# Autodesk Inventor assembly: Inner_Components
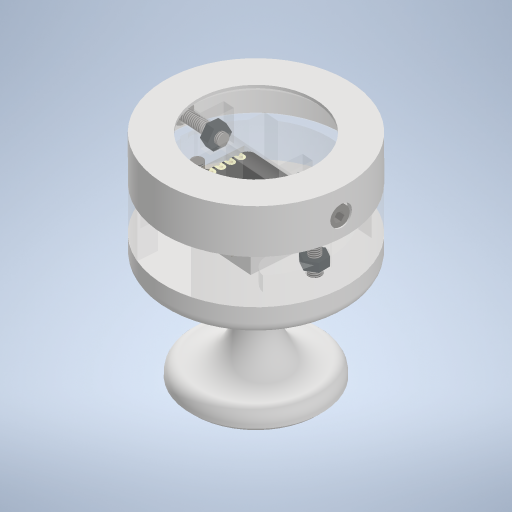
[picture p0: Inventor's stored thumbnail of the model, 512x512]
Saved by Autodesk Inventor 2023 (Build 270158000, 158)
## iProperties
Created: 2023-02-27
Part Number: Inner_Components
Document SubType Name: Assembly
Designer: maste
Author: maste
## Documents named in this file (8)
- C:\Users\maste\Documents\GitHub\Remote-Stethoscope\3D_models\ThonkLabs 1ne\SurfaceContact\Inner_Components.iam
- C:\Users\maste\Documents\GitHub\Remote-Stethoscope\3D_models\ThonkLabs 1ne\SurfaceContact\PiezoMount.ipt
- C:\Users\maste\Documents\GitHub\Remote-Stethoscope\3D_models\ThonkLabs 1ne\SurfaceContact\Piezo.ipt
- C:\Users\maste\Documents\GitHub\Remote-Stethoscope\3D_models\ThonkLabs 1ne\SurfaceContact\Diaphragm_lock.ipt
- C:\Users\maste\Documents\GitHub\Remote-Stethoscope\3D_models\ThonkLabs 1ne\SurfaceContact\holding_socket.ipt
- C:\Users\maste\Documents\GitHub\Remote-Stethoscope\3D_models\ThonkLabs 1ne\SurfaceContact\fasten_nut.ipt
- C:\Users\maste\Documents\GitHub\Remote-Stethoscope\3D_models\ThonkLabs 1ne\SurfaceContact\fasten_bolt.ipt
- C:\Users\maste\Documents\GitHub\Remote-Stethoscope\3D_models\xiao_rp2040\Seeed Studio XIAO RP2040 v26.iam
## Components (13 placed, 7 different names)
1. PiezoMount:1 — Mate:2, Mate:7, Mate:8, Mate:9, Mate:10, Mate:11, Mate:12, Mate:14, Mate:15, Mate:16, Mate:17, Mate:23, Mate:24, Mate:25, Mate:26, Mate:27, Mate:28, Mate:29, Mate:30, Mate:31, Mate:32, Mate:33, Flush:1, Mate:34
2. Piezo:1 — Mate:2, Mate:12, Mate:22
3. Diaphragm_lock:1 — Mate:11, Mate:22
4. holding_socket:1 — Mate:7, Mate:8, Mate:9, Mate:10, Mate:18, Mate:19, Mate:20, Mate:21
5. fasten_nut:1 — Mate:14, Mate:15, Mate:23
6. fasten_nut:2 — Mate:16, Mate:17, Mate:24
7. fasten_bolt:1 — Mate:18, Mate:20
8. fasten_bolt:2 — Mate:19, Mate:21
9. fasten_nut:3 — Mate:27, Mate:28
10. fasten_nut:4 — Mate:25, Mate:26
11. fasten_bolt:3 — Mate:30, Mate:31
12. fasten_bolt:4 — Mate:29, Mate:32
13. Seeed Studio XIAO RP2040 v26:1 [sub-assembly] — Mate:33, Flush:1, Mate:34
## Relationships (29: Mate 28, Flush 1)
- Mate:2: PiezoMount:1 ↔ Piezo:1
- Mate:7: PiezoMount:1 ↔ holding_socket:1
- Mate:8: PiezoMount:1 ↔ holding_socket:1
- Mate:9: PiezoMount:1 ↔ holding_socket:1
- Mate:10: PiezoMount:1 ↔ holding_socket:1
- Mate:11: PiezoMount:1 ↔ Diaphragm_lock:1
- Mate:12: PiezoMount:1 ↔ Piezo:1
- Mate:14: PiezoMount:1 ↔ fasten_nut:1
- Mate:15: PiezoMount:1 ↔ fasten_nut:1
- Mate:16: PiezoMount:1 ↔ fasten_nut:2
- Mate:17: PiezoMount:1 ↔ fasten_nut:2
- Mate:18: holding_socket:1 ↔ fasten_bolt:1
- Mate:19: holding_socket:1 ↔ fasten_bolt:2
- Mate:20: holding_socket:1 ↔ fasten_bolt:1
- Mate:21: holding_socket:1 ↔ fasten_bolt:2
- Mate:22: Piezo:1 ↔ Diaphragm_lock:1
- Mate:23: PiezoMount:1 ↔ fasten_nut:1
- Mate:24: PiezoMount:1 ↔ fasten_nut:2
- Mate:25: PiezoMount:1 ↔ fasten_nut:4
- Mate:26: PiezoMount:1 ↔ fasten_nut:4
- Mate:27: PiezoMount:1 ↔ fasten_nut:3
- Mate:28: PiezoMount:1 ↔ fasten_nut:3
- Mate:29: PiezoMount:1 ↔ fasten_bolt:4
- Mate:30: PiezoMount:1 ↔ fasten_bolt:3
- Mate:31: PiezoMount:1 ↔ fasten_bolt:3
- Mate:32: PiezoMount:1 ↔ fasten_bolt:4
- Mate:33: PiezoMount:1 ↔ Seeed Studio XIAO RP2040 v26:1
- Flush:1 (-10 mm): PiezoMount:1 ↔ Seeed Studio XIAO RP2040 v26:1
- Mate:34 (1.5 mm): PiezoMount:1 ↔ Seeed Studio XIAO RP2040 v26:1
